# Autodesk Inventor assembly: Pendulum Suspension Assembly
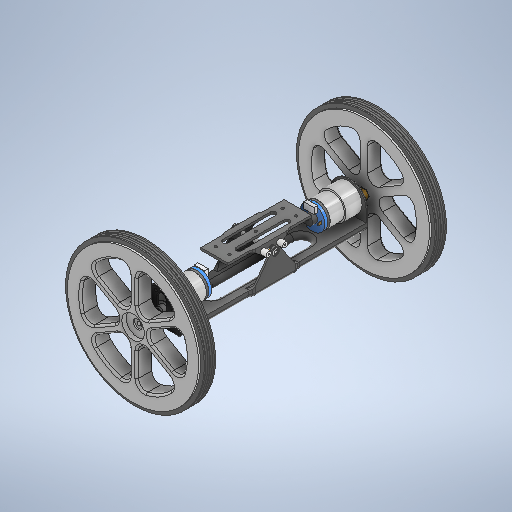
[picture p0: Inventor's stored thumbnail of the model, 512x512]
Saved by Autodesk Inventor 2025.2 (Build 292293000, 293)
## iProperties
Created: 2025-01-23
Part Number: Pendulum Suspension Assembly
Document SubType Name: Assembly
Designer: Matt Tidd
Author: Matt Tidd
## Documents named in this file (11)
- C:\Users\mtidd2\Desktop\H2A\CAD\Motors_and_Wheels\Pendulum Suspension\Pendulum Suspension Assembly.iam
- C:\Users\mtidd2\Desktop\H2A\CAD\Motors_and_Wheels\Pendulum Suspension\Pendulum Bottom Bracket.ipt
- C:\Users\mtidd2\Desktop\H2A\CAD\Motors_and_Wheels\Pendulum Suspension\Rotation Pin.ipt
- C:\Users\mtidd2\Desktop\H2A\CAD\Motors_and_Wheels\Pendulum Suspension\Rotation Bearing.ipt
- C:\Users\mtidd2\Desktop\H2A\CAD\Motors_and_Wheels\Pendulum Suspension\Rotation End Cap.ipt
- C:\Users\mtidd2\Desktop\H2A\CAD\Motors_and_Wheels\Pendulum Suspension\Pendulum Top Bracket.ipt
- C:\Users\mtidd2\Desktop\H2A\CAD\Motors_and_Wheels\520 DC Gear Motor.ipt
- C:\Users\mtidd2\Desktop\H2A\CAD\Motors_and_Wheels\Pendulum Suspension\Rotation Bumper.ipt
- C:\Users\mtidd2\Desktop\H2A\CAD\Motors_and_Wheels\Wheel Assembly\520 DC Gear Motor Wheel Coupler.ipt
- C:\Users\mtidd2\Desktop\H2A\CAD\Motors_and_Wheels\Wheel Assembly\PLA Wheel Frame.ipt
- C:\Users\mtidd2\Desktop\H2A\CAD\Motors_and_Wheels\Wheel Assembly\TPU Tire.ipt
## Components (17 placed, 10 different names)
1. Pendulum Bottom Bracket:1 — Rigid:3, Rigid:4, Rotational:1, Rotational:3, Bracket Rotation Joint
2. Rotation Pin:1 — Rotational:2
3. Rotation Bearing:1 — Rotational:4
4. Rotation End Cap:1 — Rotational:3, Rotational:5
5. Rotation Bearing:2 — Rotational:5, Rotational:6
6. Rotation End Cap:2 — Rotational:1, Rotational:2, Rotational:4
7. Pendulum Top Bracket:1 — Rigid:1, Rigid:2, Rotational:6, Bracket Rotation Joint
8. 520 DC Gear Motor:1 — Rigid:4, Rotational:8
9. 520 DC Gear Motor:2 — Rigid:3, Rotational:7
10. Rotation Bumper:1 — Rigid:2
11. Rotation Bumper:2 — Rigid:1
12. 520 DC Gear Motor Wheel Coupler:1 — Rotational:8, Rigid:6
13. 520 DC Gear Motor Wheel Coupler:2 — Rotational:7, Rigid:5
14. PLA Wheel Frame:1 — Rigid:6, Rigid:7
15. PLA Wheel Frame:2 — Rigid:5, Rigid:8
16. TPU Tire:1 — Rigid:7
17. TPU Tire:2 — Rigid:8
## Relationships (17: RevoluteJoint 9, WeldJoint 8)
- Rigid:1 [WeldJoint]: Pendulum Top Bracket:1 ↔ Rotation Bumper:2
- Rigid:2 [WeldJoint]: Pendulum Top Bracket:1 ↔ Rotation Bumper:1
- Rigid:3 [WeldJoint]: Pendulum Bottom Bracket:1 ↔ 520 DC Gear Motor:2
- Rigid:4 [WeldJoint]: Pendulum Bottom Bracket:1 ↔ 520 DC Gear Motor:1
- Rotational:1 [RevoluteJoint]: Pendulum Bottom Bracket:1 ↔ Rotation End Cap:2
- Rotational:2 [RevoluteJoint]: Rotation Pin:1 ↔ Rotation End Cap:2
- Rotational:3 [RevoluteJoint]: Pendulum Bottom Bracket:1 ↔ Rotation End Cap:1
- Rotational:4 [RevoluteJoint]: Rotation Bearing:1 ↔ Rotation End Cap:2
- Rotational:5 [RevoluteJoint]: Rotation End Cap:1 ↔ Rotation Bearing:2
- Rotational:6 [RevoluteJoint]: Rotation Bearing:2 ↔ Pendulum Top Bracket:1
- Rotational:7 [RevoluteJoint]: 520 DC Gear Motor:2 ↔ 520 DC Gear Motor Wheel Coupler:2
- Rotational:8 [RevoluteJoint]: 520 DC Gear Motor:1 ↔ 520 DC Gear Motor Wheel Coupler:1
- Rigid:5 [WeldJoint]: 520 DC Gear Motor Wheel Coupler:2 ↔ PLA Wheel Frame:2
- Rigid:6 [WeldJoint]: 520 DC Gear Motor Wheel Coupler:1 ↔ PLA Wheel Frame:1
- Rigid:7 [WeldJoint]: PLA Wheel Frame:1 ↔ TPU Tire:1
- Rigid:8 [WeldJoint]: PLA Wheel Frame:2 ↔ TPU Tire:2
- Bracket Rotation Joint [RevoluteJoint] (-8 mm): Pendulum Bottom Bracket:1 ↔ Pendulum Top Bracket:1
